# Autodesk Inventor assembly: 04-00-Привод передний
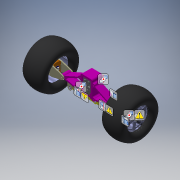
[picture p0: Inventor's stored thumbnail of the model, 180x180]
Saved by Autodesk Inventor 2018 (Build 220112000, 112)
## iProperties
Part Number: 04-00-Привод передний
Material: Типовые
Document SubType Name: Assembly
Designer: sbnnl
Author: sbnnl
## Documents named in this file (15)
- D:\Загрузки\IMMO\04-00-Привод передний.iam
- D:\Загрузки\IMMO\01-00-Колесо.iam
- D:\Загрузки\IMMO\04-03-Ось.ipt
- D:\Загрузки\IMMO\04-04-Кулак.ipt
- D:\Загрузки\IMMO\Крепеж\Гайка М10.ipt
- D:\Загрузки\IMMO\Подшипники\Подшипник 6х19.ipt
- D:\Загрузки\IMMO\Крепеж\Гайка М6.ipt
- D:\Загрузки\IMMO\04-06-Рычаг.ipt
- D:\Загрузки\IMMO\04-07-Коромысло правое.ipt
- D:\Загрузки\IMMO\04-07-Коромысло левое.ipt
- D:\Загрузки\IMMO\04-08-Опора.ipt
- D:\Загрузки\IMMO\04-02-Тяга.ipt
- D:\Загрузки\IMMO\Подшипники\Подшипник 4х8-Ю.ipt
- D:\Загрузки\IMMO\Dynamixel AX-12\AX-12A.iam
- D:\Загрузки\IMMO\04-01-Качалка.ipt
## Components (31 placed, 14 different names)
1. 01-00-Колесо:1 [sub-assembly] — Совмещение:1, Совмещение:2, Совмещение:4, Совмещение:5
2. Гайка М10:1 — Совмещение:1, Совмещение:2, Совмещение:3, Заподлицо:1, Совмещение:6, Заподлицо:2
3. Гайка М10:2 — Совмещение:3, Заподлицо:1, Совмещение:4, Совмещение:5
4. Подшипник 6х19:1 — Совмещение:7, Совмещение:10, Совмещение:12, Совмещение:13
5. Подшипник 6х19:2 — Совмещение:8, Совмещение:9, Совмещение:11, Совмещение:14
6. 04-03-Ось:1 — Совмещение:6, Заподлицо:2, Совмещение:7, Совмещение:8, Совмещение:13, Совмещение:15
7. 04-04-Кулак:1 — Совмещение:9, Совмещение:10, Совмещение:11, Совмещение:12, Совмещение:16, Совмещение:17, Совмещение:18, Совмещение:19, Совмещение:20, Совмещение:21
8. Гайка М6:1 — Совмещение:14, Совмещение:15
9. 04-06-Рычаг:1 — Совмещение:16, Совмещение:17, Совмещение:18
10. 04-07-Коромысло правое:1 — Совмещение:19, Совмещение:20, Совмещение:21, С поворотом:6, С поворотом:8
11. 01-00-Колесо:2 [sub-assembly] — Совмещение:22, Совмещение:24, Цилиндрический:2
12. Гайка М10:3 — Совмещение:22, Жесткий:1
13. Гайка М10:4 — Совмещение:24, Цилиндрический:1
14. Подшипник 6х19:3 — Совмещение:27, Совмещение:29, Совмещение:31, Совмещение:33
15. Подшипник 6х19:4 — Совмещение:28, Совмещение:32, Совмещение:34, Совмещение:36
16. 04-03-Ось:2 — Совмещение:27, Совмещение:28, Совмещение:29, Совмещение:35, Цилиндрический:1, Цилиндрический:2, Жесткий:1
17. 04-04-Кулак:2 — Совмещение:31, Совмещение:32, Совмещение:33, Совмещение:34, Совмещение:37, Совмещение:38, Совмещение:39, Совмещение:40, Совмещение:41, Совмещение:42
18. Гайка М6:2 — Совмещение:35, Совмещение:36
19. 04-06-Рычаг:2 — Совмещение:37, Совмещение:38, Совмещение:39
20. 04-07-Коромысло левое:1 — Совмещение:40, Совмещение:41, Совмещение:42, Совмещение:86, Совмещение:95, С поворотом:5, Совмещение:96, С поворотом:7
21. 04-08-Опора:1 — С поворотом:1, С поворотом:2, С поворотом:3, С поворотом:4, Совмещение:97, Совмещение:98
22. 04-02-Тяга:1 — Совмещение:71, Совмещение:72, Совмещение:73, Заподлицо:6, Совмещение:77, С поворотом:12
23. Подшипник 4х8-Ю:1 — Совмещение:71, Совмещение:72, С поворотом:7
24. Подшипник 4х8-Ю:2 — Совмещение:73, Совмещение:77, С поворотом:8
25. Подшипник 4х8-Ю:3 — Заподлицо:6, С поворотом:10, С поворотом:12
26. Подшипник 4х8-Ю:4 — Совмещение:86, Совмещение:95, С поворотом:1, С поворотом:5, Совмещение:96
27. Подшипник 4х8-Ю:5 — С поворотом:3
28. Подшипник 4х8-Ю:6 — С поворотом:2
29. Подшипник 4х8-Ю:7 — С поворотом:4, С поворотом:6
30. AX-12A:1 [sub-assembly] — Совмещение:97, Совмещение:98, С поворотом:11
31. 04-01-Качалка:1 — С поворотом:10, С поворотом:11
## Relationships (64: Mate 47, RevoluteJoint 11, Flush 3, CylindricalJoint 2, WeldJoint 1)
- Совмещение:1 [Mate]: 01-00-Колесо:1 ↔ Гайка М10:1
- Совмещение:2 [Mate]: 01-00-Колесо:1 ↔ Гайка М10:1
- Совмещение:3 [Mate]: Гайка М10:1 ↔ Гайка М10:2
- Заподлицо:1 [Flush]: Гайка М10:1 ↔ Гайка М10:2
- Совмещение:4 [Mate]: 01-00-Колесо:1 ↔ Гайка М10:2
- Совмещение:5 [Mate]: 01-00-Колесо:1 ↔ Гайка М10:2
- Совмещение:6 [Mate]: Гайка М10:1 ↔ 04-03-Ось:1
- Заподлицо:2 [Flush]: Гайка М10:1 ↔ 04-03-Ось:1
- Совмещение:7 [Mate]: Подшипник 6х19:1 ↔ 04-03-Ось:1
- Совмещение:8 [Mate]: Подшипник 6х19:2 ↔ 04-03-Ось:1
- Совмещение:9 [Mate]: Подшипник 6х19:2 ↔ 04-04-Кулак:1
- Совмещение:10 [Mate]: Подшипник 6х19:1 ↔ 04-04-Кулак:1
- Совмещение:11 [Mate]: Подшипник 6х19:2 ↔ 04-04-Кулак:1
- Совмещение:12 [Mate]: Подшипник 6х19:1 ↔ 04-04-Кулак:1
- Совмещение:13 [Mate]: Подшипник 6х19:1 ↔ 04-03-Ось:1
- Совмещение:14 [Mate]: Подшипник 6х19:2 ↔ Гайка М6:1
- Совмещение:15 [Mate]: 04-03-Ось:1 ↔ Гайка М6:1
- Совмещение:16 [Mate]: 04-04-Кулак:1 ↔ 04-06-Рычаг:1
- Совмещение:17 [Mate]: 04-04-Кулак:1 ↔ 04-06-Рычаг:1
- Совмещение:18 [Mate]: 04-04-Кулак:1 ↔ 04-06-Рычаг:1
- Совмещение:19 [Mate]: 04-04-Кулак:1 ↔ 04-07-Коромысло правое:1
- Совмещение:20 [Mate]: 04-04-Кулак:1 ↔ 04-07-Коромысло правое:1
- Совмещение:21 [Mate]: 04-04-Кулак:1 ↔ 04-07-Коромысло правое:1
- Совмещение:22 [Mate]: 01-00-Колесо:2 ↔ Гайка М10:3
- Совмещение:24 [Mate]: 01-00-Колесо:2 ↔ Гайка М10:4
- Совмещение:27 [Mate]: Подшипник 6х19:3 ↔ 04-03-Ось:2
- Совмещение:28 [Mate]: Подшипник 6х19:4 ↔ 04-03-Ось:2
- Совмещение:29 [Mate]: Подшипник 6х19:3 ↔ 04-03-Ось:2
- Совмещение:31 [Mate]: Подшипник 6х19:3 ↔ 04-04-Кулак:2
- Совмещение:32 [Mate]: Подшипник 6х19:4 ↔ 04-04-Кулак:2
- Совмещение:33 [Mate]: Подшипник 6х19:3 ↔ 04-04-Кулак:2
- Совмещение:34 [Mate]: Подшипник 6х19:4 ↔ 04-04-Кулак:2
- Совмещение:35 [Mate]: 04-03-Ось:2 ↔ Гайка М6:2
- Совмещение:36 [Mate]: Подшипник 6х19:4 ↔ Гайка М6:2
- Совмещение:37 [Mate]: 04-04-Кулак:2 ↔ 04-06-Рычаг:2
- Совмещение:38 [Mate]: 04-04-Кулак:2 ↔ 04-06-Рычаг:2
- Совмещение:39 [Mate]: 04-04-Кулак:2 ↔ 04-06-Рычаг:2
- Совмещение:40 [Mate]: 04-04-Кулак:2 ↔ 04-07-Коромысло левое:1
- Совмещение:41 [Mate]: 04-04-Кулак:2 ↔ 04-07-Коромысло левое:1
- Совмещение:42 [Mate]: 04-04-Кулак:2 ↔ 04-07-Коромысло левое:1
- Совмещение:71 [Mate]: 04-02-Тяга:1 ↔ Подшипник 4х8-Ю:1
- Совмещение:72 [Mate]: 04-02-Тяга:1 ↔ Подшипник 4х8-Ю:1
- Совмещение:73 [Mate]: 04-02-Тяга:1 ↔ Подшипник 4х8-Ю:2
- Заподлицо:6 [Flush]: 04-02-Тяга:1 ↔ Подшипник 4х8-Ю:3
- Совмещение:77 [Mate]: 04-02-Тяга:1 ↔ Подшипник 4х8-Ю:2
- Совмещение:86 [Mate]: 04-07-Коромысло левое:1 ↔ Подшипник 4х8-Ю:4
- Совмещение:95 [Mate]: 04-07-Коромысло левое:1 ↔ Подшипник 4х8-Ю:4
- С поворотом:1 [RevoluteJoint]: 04-08-Опора:1 ↔ Подшипник 4х8-Ю:4
- С поворотом:2 [RevoluteJoint]: 04-08-Опора:1 ↔ Подшипник 4х8-Ю:6
- С поворотом:3 [RevoluteJoint]: 04-08-Опора:1 ↔ Подшипник 4х8-Ю:5
- С поворотом:4 [RevoluteJoint]: 04-08-Опора:1 ↔ Подшипник 4х8-Ю:7
- С поворотом:5 [RevoluteJoint]: 04-07-Коромысло левое:1 ↔ Подшипник 4х8-Ю:4
- Совмещение:96 [Mate]: 04-07-Коромысло левое:1 ↔ Подшипник 4х8-Ю:4
- Цилиндрический:1 [CylindricalJoint]: Гайка М10:4 ↔ 04-03-Ось:2
- Цилиндрический:2 [CylindricalJoint]: 01-00-Колесо:2 ↔ 04-03-Ось:2
- Жесткий:1 [WeldJoint]: Гайка М10:3 ↔ 04-03-Ось:2
- С поворотом:6 [RevoluteJoint]: 04-07-Коромысло правое:1 ↔ Подшипник 4х8-Ю:7
- С поворотом:7 [RevoluteJoint]: 04-07-Коромысло левое:1 ↔ Подшипник 4х8-Ю:1
- С поворотом:8 [RevoluteJoint]: 04-07-Коромысло правое:1 ↔ Подшипник 4х8-Ю:2
- С поворотом:10 [RevoluteJoint]: Подшипник 4х8-Ю:3 ↔ 04-01-Качалка:1
- Совмещение:97 [Mate]: 04-08-Опора:1 ↔ AX-12A:1
- Совмещение:98 [Mate]: 04-08-Опора:1 ↔ AX-12A:1
- С поворотом:11 [RevoluteJoint]: AX-12A:1 ↔ 04-01-Качалка:1
- С поворотом:12 [RevoluteJoint]: 04-02-Тяга:1 ↔ Подшипник 4х8-Ю:3
